# Autodesk Inventor assembly: DualJagSettup
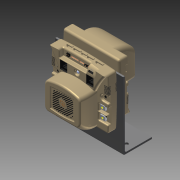
[picture p0: Inventor's stored thumbnail of the model, 180x180]
Saved by Autodesk Inventor 2012 (Build 160160000, 160)
## iProperties
Created: 2012-01-11
Part Number: DualJagSettup
Document SubType Name: Assembly
Designer: William
Author: William
## Documents named in this file (3)
- C:\Users\William\Dropbox\Robotics\CAD\team1885frc\Robot2012\Concepts\Electronics Board\DualJagSettup.iam
- C:\Users\William\Dropbox\Robotics\CAD\team1885frc\Electronics\dualjaguarstand.ipt
- C:\Users\William\Dropbox\Robotics\CAD\team1885frc\Electronics\Jag\Jag.iam
## Components (3 placed, 2 different names)
1. dualjaguarstand:1 — Mate:1, Mate:2, Mate:3, Mate:4, Angle:1, Angle:2
2. Jag:1 [sub-assembly] — Mate:1, Mate:2, Angle:2
3. Jag:2 [sub-assembly] — Mate:3, Mate:4, Angle:1
## Relationships (6: Mate 4, Angle 2)
- Mate:1: dualjaguarstand:1 ↔ Jag:1
- Mate:2: dualjaguarstand:1 ↔ Jag:1
- Mate:3: dualjaguarstand:1 ↔ Jag:2
- Mate:4: dualjaguarstand:1 ↔ Jag:2
- Angle:1 (0 deg): dualjaguarstand:1 ↔ Jag:2
- Angle:2 (0 deg): dualjaguarstand:1 ↔ Jag:1
